# Autodesk Inventor assembly: Assembly1
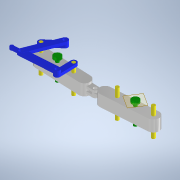
[picture p0: Inventor's stored thumbnail of the model, 180x180]
Saved by Autodesk Inventor 2022 (Build 260153000, 153)
## iProperties
Created: 2022-02-01
Part Number: Assembly1
Document SubType Name: Assembly
Designer: br4ch
Author: br4ch
## Documents named in this file (9)
- C:\Users\br4ch\M-and-Ms\Legs\Assembly1.iam
- C:\Users\br4ch\M-and-Ms\Legs\Part5.ipt
- C:\Users\br4ch\M-and-Ms\Legs\Part6.ipt
- C:\Users\br4ch\M-and-Ms\Legs\Part7.ipt
- C:\Users\br4ch\M-and-Ms\Legs\Part8.ipt
- C:\Users\br4ch\M-and-Ms\Legs\Part9.ipt
- C:\Users\br4ch\M-and-Ms\Legs\Part10.ipt
- C:\Users\br4ch\M-and-Ms\Legs\Assembly1\Design Accelerator\front gears1.iam
- C:\Users\br4ch\M-and-Ms\Legs\Shaft1.ipt
## Components (14 placed, 8 different names)
1. Part5:1 — Rotational:4, Rotational:11
2. Part6:1 — Rotational:4, Rotational:13
3. Part7:1 — Rotational:10, Rotational:17, Rotational:18, Rotational:23
4. Part8:1 — Rotational:10, Rotational:14, Rotational:16, Rotational:20
5. Part5:2 — Rotational:9, Rotational:12
6. Part9:1 — Rotational:12, Rotational:13
7. Part10:1 — Rotational:14, Rotational:11
8. Part10:3 — Rotational:16, Rotational:9
9. Part10:4 — Rotational:17
10. Part10:6 — Rotational:18
11. front gears:1 [sub-assembly] — Rotational:21
12. Shaft:1 — Rotational:20, Rotational:21
13. front gears:2 [sub-assembly] — Flush:1, Symmetry:1
14. Shaft:2 — Rotational:23
## Relationships (16: RevoluteJoint 14, Flush 1, Symmetry 1)
- Rotational:4 [RevoluteJoint]: Part5:1 ↔ Part6:1
- Rotational:9 [RevoluteJoint]: Part5:2 ↔ Part10:3
- Rotational:10 [RevoluteJoint]: Part7:1 ↔ Part8:1
- Rotational:11 [RevoluteJoint]: Part5:1 ↔ Part10:1
- Rotational:12 [RevoluteJoint]: Part5:2 ↔ Part9:1
- Rotational:13 [RevoluteJoint]: Part6:1 ↔ Part9:1
- Rotational:14 [RevoluteJoint]: Part8:1 ↔ Part10:1
- Rotational:16 [RevoluteJoint]: Part8:1 ↔ Part10:3
- Rotational:17 [RevoluteJoint]: Part7:1 ↔ Part10:4
- Rotational:18 [RevoluteJoint]: Part7:1 ↔ Part10:6
- Rotational:20 [RevoluteJoint]: Part8:1 ↔ Shaft:1
- Rotational:21 [RevoluteJoint]: front gears:1 ↔ Shaft:1
- [RevoluteJoint]: front gears:2 ↔ Shaft:2
- Rotational:23 [RevoluteJoint]: Part7:1 ↔ Shaft:2
- Flush:1: front gears:2
- Symmetry:1: front gears:2
## Named parameters: th = 5 mm, r = 6 mm, R = 10 mm, w = 20 mm, d48_d47 = 155.883082 deg, d49_d46 = 0 mm
